# Autodesk Inventor assembly: CompositeSupport-3
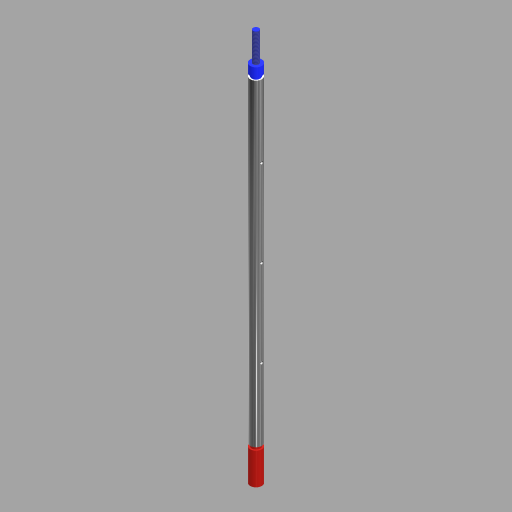
[picture p0: Inventor's stored thumbnail of the model, 512x512]
Saved by Autodesk Inventor 2024 (Build 280153020, 153B)
## iProperties
Created: 2023-09-24
Part Number: CompositeSupport-3
Document SubType Name: Assembly
Designer: schanen
Author: schanen
## Documents named in this file (4)
- C:\Users\schanen\Documents\Inventor\he4inserts\CompositeSupport-3.iam
- C:\Users\schanen\Documents\Inventor\he4inserts\Fitting-1.ipt
- C:\Users\schanen\Documents\Inventor\he4inserts\Fitting-2.ipt
- C:\Users\schanen\Documents\Inventor\he4inserts\InsertTube4OD0.5W120L.ipt
## Components (3 placed, 3 different names)
1. Fitting-1:1
2. Fitting-2:1
3. InsertTube4OD0.5W120L:1
## Relationships (4: Mate 4)
- [Mate]: Fitting-1:1 ↔ InsertTube4OD0.5W120L:1
- [Mate]: Fitting-2:1 ↔ InsertTube4OD0.5W120L:1
- [Mate] (1 mm): Fitting-1:1 ↔ InsertTube4OD0.5W120L:1
- [Mate] (1 mm): Fitting-2:1 ↔ InsertTube4OD0.5W120L:1
